# Autodesk Inventor assembly: cORTE_PERFIL
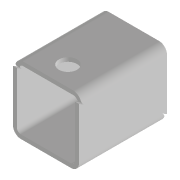
[picture p0: Inventor's stored thumbnail of the model, 180x180]
Saved by Autodesk Inventor 2020 (Build 240168000, 168)
## iProperties
Created: 2020-03-03
Part Number: cORTE_PERFIL
Document SubType Name: Assembly
Designer: Juan Carlos Botero
Author: Juan Carlos Botero
## Documents named in this file (2)
- D:\Drives\OneDrive\Carlos_2\02 TRABAJOS\MULTIPLO\Conveyor\ENSAMBLE - Copy\cORTE_PERFIL.iam
- D:\Drives\OneDrive\Carlos_2\02 TRABAJOS\MULTIPLO\Conveyor\ENSAMBLE - Copy\Soporte Fijo.ipt
## Components (2 placed, 1 different names)
1. Soporte Fijo:1 — Mate:1, Flush:1, Mate:2
2. Soporte Fijo:2 — Mate:1, Flush:1, Mate:2
## Relationships (3: Mate 2, Flush 1)
- Mate:1: Soporte Fijo:1 ↔ Soporte Fijo:2
- Flush:1: Soporte Fijo:1 ↔ Soporte Fijo:2
- Mate:2 (-50 mm): Soporte Fijo:1 ↔ Soporte Fijo:2
